# Autodesk Inventor assembly: PRTGN_Assembly
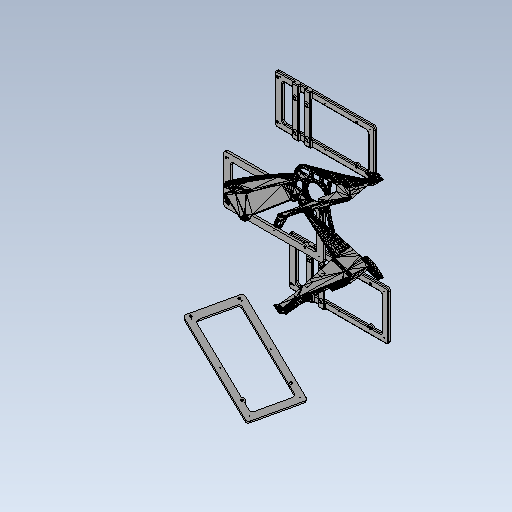
[picture p0: Inventor's stored thumbnail of the model, 512x512]
Saved by Autodesk Inventor 2026.2 (Build 302298000, 298)
## iProperties
Created: 2026-05-31
Part Number: PRTGN_Assembly
Document SubType Name: Assembly
Designer: MenMe
Author: MenMe
## Documents named in this file (4)
- C:\Users\MenMe\GitHub\PRTGN\Mechanics\PRTGN_Assembly\PRTGN_Assembly.iam
- C:\Users\MenMe\Downloads\DisplayMountJtingf\electronics_mount v2.ipt
- C:\Users\MenMe\GitHub\PRTGN\Mechanics\PRTGN_Assembly\display_mount_inner\display_mount_inner\display_mount_inner.ipt
- C:\Users\MenMe\GitHub\PRTGN\Mechanics\PRTGN_Assembly\display_mount_outer\display_mount_outer\display_mount_outer.ipt
## Components (5 placed, 3 different names)
1. electronics_mount v2:1 — Mate:1
2. display_mount_inner:1
3. display_mount_outer:1
4. display_mount_outer:2 — Mate:1
5. display_mount_inner:2
## Relationships (1: Mate 1)
- Mate:1: electronics_mount v2:1 ↔ display_mount_outer:2
